# Autodesk Inventor assembly: Assembly
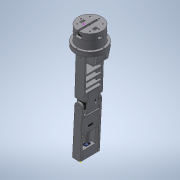
[picture p0: Inventor's stored thumbnail of the model, 180x180]
Saved by Autodesk Inventor 2020.1 (Build 241239000, 239)
## iProperties
Created: 2017-12-03
Part Number: Assembly
Document SubType Name: Assembly
Designer: Bardo91
Author: Bardo91
## Documents named in this file (16)
- D:\programming\hecatonquiros\cad_models\arm_4_dof\serial_model\Assembly.iam
- D:\programming\hecatonquiros\cad_models\arm_4_dof\serial_model\arm_0_attachment.ipt
- D:\programming\hecatonquiros\cad_models\arm_4_dof\serial_model\arm_0_top.ipt
- D:\programming\hecatonquiros\cad_models\arm_4_dof\serial_model\servo_FT_SC.ipt
- D:\programming\hecatonquiros\cad_models\arm_4_dof\serial_model\arm_0_bottom.ipt
- D:\programming\hecatonquiros\cad_models\arm_4_dof\serial_model\arm_0_bottom_top_lock.ipt
- D:\programming\hecatonquiros\cad_models\arm_4_dof\serial_model\servo_FT_SC_horn_1.ipt
- D:\programming\hecatonquiros\cad_models\arm_4_dof\serial_model\arm_0_bottom_case.ipt
- D:\programming\hecatonquiros\cad_models\arm_4_dof\serial_model\servo_FT_SC_horn_2.ipt
- D:\programming\hecatonquiros\cad_models\arm_4_dof\serial_model\arm_1.ipt
- D:\programming\hecatonquiros\cad_models\arm_4_dof\serial_model\arm_1_case.ipt
- D:\programming\hecatonquiros\cad_models\arm_4_dof\serial_model\arm_2_case_bearing.ipt
- D:\programming\hecatonquiros\cad_models\arm_4_dof\serial_model\bearing.ipt
- D:\programming\hecatonquiros\cad_models\arm_4_dof\serial_model\arm_2_case.ipt
- D:\programming\hecatonquiros\cad_models\arm_4_dof\serial_model\arm_2.ipt
- D:\programming\hecatonquiros\cad_models\arm_4_dof\serial_model\end_effector_connector_arm2_grande.ipt
## Components (23 placed, 15 different names)
1. arm_0_attachment:1 — Mate:1, Mate:2, Mate:3
2. arm_0_top:1 — Mate:1, Mate:2, Mate:3, Mate:4, Mate:5, Mate:6, Mate:7, Flush:1
3. servo_FT_SC:1 — Mate:4, Mate:5, Mate:6, Mate:18
4. servo_FT_SC_horn_1:1 — Mate:18, Mate:19, Mate:20
5. arm_0_bottom:1 — Mate:7, Flush:1, Mate:14, Mate:15, Mate:16, Mate:19, Mate:20, Mate:21, Mate:22, Mate:23, Mate:24, Mate:25, Mate:26, Mate:27
6. arm_0_bottom_top_lock:1 — Mate:14, Mate:15, Mate:16
7. servo_FT_SC:2 — Mate:21, Mate:22, Mate:23, Mate:28, Mate:29, Mate:34
8. arm_0_bottom_case:1 — Mate:24, Mate:25, Mate:26, Mate:27
9. servo_FT_SC_horn_1:2 — Mate:28, Mate:29, Mate:31, Mate:32, Mate:33
10. arm_1:1 — Mate:31, Mate:32, Mate:33, Mate:35, Mate:36, Mate:37, Mate:38, Mate:39, Mate:40, Mate:41, Mate:42
11. servo_FT_SC_horn_2:1 — Mate:34, Mate:35, Mate:36
12. servo_FT_SC:3 — Mate:37, Mate:38, Mate:39, Coincidencia:44, Coincidencia:45, Mate:64
13. arm_1_case:1 — Mate:40, Mate:41, Mate:42
14. servo_FT_SC_horn_1:3 — Coincidencia:44, Coincidencia:45, Mate:46, Mate:47, Mate:48
15. bearing:1 — Mate:50, Mate:52
16. bearing:2 — Mate:49, Mate:51
17. arm_2_case:1 — Mate:55, Mate:56, Mate:58
18. arm_2_case_bearing:1 — Mate:53, Mate:54, Mate:57
19. arm_2:1 — Mate:46, Mate:47, Mate:48, Mate:49, Mate:50, Mate:51, Mate:52, Mate:53, Mate:54, Mate:55, Mate:56, Mate:57, Mate:58, Mate:59, Mate:60, Mate:61, Mate:65, Mate:66
20. servo_FT_SC:4 — Mate:59, Mate:60, Mate:61, Mate:62, Mate:63
21. servo_FT_SC_horn_2:2 — Mate:64, Mate:65, Mate:66
22. servo_FT_SC_horn_1:4 — Mate:62, Mate:63, Mate:67, Mate:68, Mate:69
23. end_effector_connector_arm2_grande:1 — Mate:67, Mate:68, Mate:69
## Relationships (61: Mate 60, Flush 1)
- Mate:1: arm_0_attachment:1 ↔ arm_0_top:1
- Mate:2: arm_0_attachment:1 ↔ arm_0_top:1
- Mate:3: arm_0_attachment:1 ↔ arm_0_top:1
- Mate:4: arm_0_top:1 ↔ servo_FT_SC:1
- Mate:5: arm_0_top:1 ↔ servo_FT_SC:1
- Mate:6: arm_0_top:1 ↔ servo_FT_SC:1
- Mate:7: arm_0_top:1 ↔ arm_0_bottom:1
- Flush:1: arm_0_top:1 ↔ arm_0_bottom:1
- Mate:14: arm_0_bottom:1 ↔ arm_0_bottom_top_lock:1
- Mate:15: arm_0_bottom:1 ↔ arm_0_bottom_top_lock:1
- Mate:16: arm_0_bottom:1 ↔ arm_0_bottom_top_lock:1
- Mate:18: servo_FT_SC:1 ↔ servo_FT_SC_horn_1:1
- Mate:19: servo_FT_SC_horn_1:1 ↔ arm_0_bottom:1
- Mate:20: servo_FT_SC_horn_1:1 ↔ arm_0_bottom:1
- Mate:21: arm_0_bottom:1 ↔ servo_FT_SC:2
- Mate:22: arm_0_bottom:1 ↔ servo_FT_SC:2
- Mate:23: arm_0_bottom:1 ↔ servo_FT_SC:2
- Mate:24: arm_0_bottom:1 ↔ arm_0_bottom_case:1
- Mate:25: arm_0_bottom:1 ↔ arm_0_bottom_case:1
- Mate:26: arm_0_bottom:1 ↔ arm_0_bottom_case:1
- Mate:27: arm_0_bottom:1 ↔ arm_0_bottom_case:1
- Mate:28: servo_FT_SC:2 ↔ servo_FT_SC_horn_1:2
- Mate:29: servo_FT_SC:2 ↔ servo_FT_SC_horn_1:2
- Mate:31: servo_FT_SC_horn_1:2 ↔ arm_1:1
- Mate:32: servo_FT_SC_horn_1:2 ↔ arm_1:1
- Mate:33: servo_FT_SC_horn_1:2 ↔ arm_1:1
- Mate:34: servo_FT_SC:2 ↔ servo_FT_SC_horn_2:1
- Mate:35: arm_1:1 ↔ servo_FT_SC_horn_2:1
- Mate:36: arm_1:1 ↔ servo_FT_SC_horn_2:1
- Mate:37: arm_1:1 ↔ servo_FT_SC:3
- Mate:38: arm_1:1 ↔ servo_FT_SC:3
- Mate:39: arm_1:1 ↔ servo_FT_SC:3
- Mate:40: arm_1:1 ↔ arm_1_case:1
- Mate:41: arm_1:1 ↔ arm_1_case:1
- Mate:42: arm_1:1 ↔ arm_1_case:1
- Coincidencia:44 [Mate]: servo_FT_SC:3 ↔ servo_FT_SC_horn_1:3
- Coincidencia:45 [Mate]: servo_FT_SC:3 ↔ servo_FT_SC_horn_1:3
- Mate:46: servo_FT_SC_horn_1:3 ↔ arm_2:1
- Mate:47: servo_FT_SC_horn_1:3 ↔ arm_2:1
- Mate:48: servo_FT_SC_horn_1:3 ↔ arm_2:1
- Mate:49: bearing:2 ↔ arm_2:1
- Mate:50: bearing:1 ↔ arm_2:1
- Mate:51: bearing:2 ↔ arm_2:1
- Mate:52: bearing:1 ↔ arm_2:1
- Mate:53: arm_2_case_bearing:1 ↔ arm_2:1
- Mate:54: arm_2_case_bearing:1 ↔ arm_2:1
- Mate:55: arm_2_case:1 ↔ arm_2:1
- Mate:56: arm_2_case:1 ↔ arm_2:1
- Mate:57: arm_2_case_bearing:1 ↔ arm_2:1
- Mate:58: arm_2_case:1 ↔ arm_2:1
- Mate:59: arm_2:1 ↔ servo_FT_SC:4
- Mate:60: arm_2:1 ↔ servo_FT_SC:4
- Mate:61: arm_2:1 ↔ servo_FT_SC:4
- Mate:62: servo_FT_SC:4 ↔ servo_FT_SC_horn_1:4
- Mate:63: servo_FT_SC:4 ↔ servo_FT_SC_horn_1:4
- Mate:64: servo_FT_SC:3 ↔ servo_FT_SC_horn_2:2
- Mate:65: arm_2:1 ↔ servo_FT_SC_horn_2:2
- Mate:66: arm_2:1 ↔ servo_FT_SC_horn_2:2
- Mate:67: servo_FT_SC_horn_1:4 ↔ end_effector_connector_arm2_grande:1
- Mate:68: servo_FT_SC_horn_1:4 ↔ end_effector_connector_arm2_grande:1
- Mate:69: servo_FT_SC_horn_1:4 ↔ end_effector_connector_arm2_grande:1
